# Autodesk Inventor assembly: Extruder Midbody Assembly
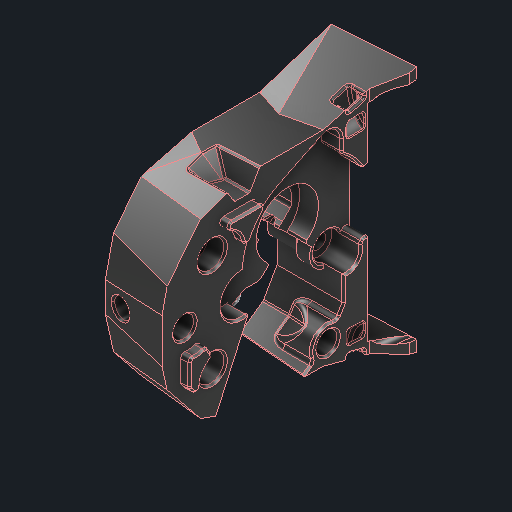
[picture p0: Inventor's stored thumbnail of the model, 512x512]
Saved by Autodesk Inventor 2025.1 (Build 291241020, 241B)
## iProperties
Created: 2025-05-11
Part Number: Extruder Midbody Assembly
Document SubType Name: Assembly
Designer: Joshua Eah
Author: Joshua Eah
## Documents named in this file (3)
- C:\Users\Joshua Eah\Documents\Voron 0.2\CAD\Master Assembly\Toolhead\Extruder Midbody Assembly.iam
- C:\Users\Joshua Eah\Documents\Voron 0.2\CAD\Master Assembly\Hardware\M2x6 FHCS.ipt
- C:\Users\Joshua Eah\Documents\Voron 0.2\CAD\Master Assembly\Extriuder Midbody.ipt
## Components (2 placed, 2 different names)
1. M2x6 FHCS:1 — Mate:1
2. Extruder Midbody:1 — Mate:1
## Relationships (1: Mate 1)
- Mate:1: M2x6 FHCS:1 ↔ Extruder Midbody:1
